# Autodesk Inventor assembly: main
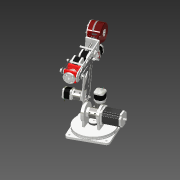
[picture p0: Inventor's stored thumbnail of the model, 180x180]
Saved by Autodesk Inventor 2020 (Build 240168000, 168)
## iProperties
Created: 2020-05-24
Part Number: main
Document SubType Name: Assembly
Designer: Svend
Author: Svend
## Documents named in this file (5)
- D:\github_gedeeld\BeerMinder\3D-model\mainAssembly\main.iam
- D:\github_gedeeld\BeerMinder\3D-model\axis4\axis4.iam
- D:\github_gedeeld\BeerMinder\3D-model\axis3\axis3.iam
- D:\github_gedeeld\BeerMinder\3D-model\Base (Axis 1)\gefreesd\AssemblyGefreesdBasev2.iam
- D:\github_gedeeld\BeerMinder\3D-model\axis5_6\axis5_6  compact.iam
## Components (4 placed, 4 different names)
1. axis4:1 [sub-assembly] — Mate:5, Mate:6, Mate:7, Mate:8
2. axis3:1 [sub-assembly] — Mate:3, Mate:4, Mate:5, Mate:6
3. AssemblyGefreesdBasev2:1 [sub-assembly] — Mate:1, Mate:2, Flush:1, Mate:3, Mate:4
4. axis5_6  compact:1 [sub-assembly] — Mate:7, Mate:8
## Relationships (9: Mate 8, Flush 1)
- Mate:1: AssemblyGefreesdBasev2:1
- Mate:2: AssemblyGefreesdBasev2:1
- Flush:1: AssemblyGefreesdBasev2:1
- Mate:3: axis3:1 ↔ AssemblyGefreesdBasev2:1
- Mate:4: axis3:1 ↔ AssemblyGefreesdBasev2:1
- Mate:5: axis4:1 ↔ axis3:1
- Mate:6: axis4:1 ↔ axis3:1
- Mate:7: axis4:1 ↔ axis5_6  compact:1
- Mate:8 (1 mm): axis4:1 ↔ axis5_6  compact:1
